# Autodesk Inventor assembly: Tolva
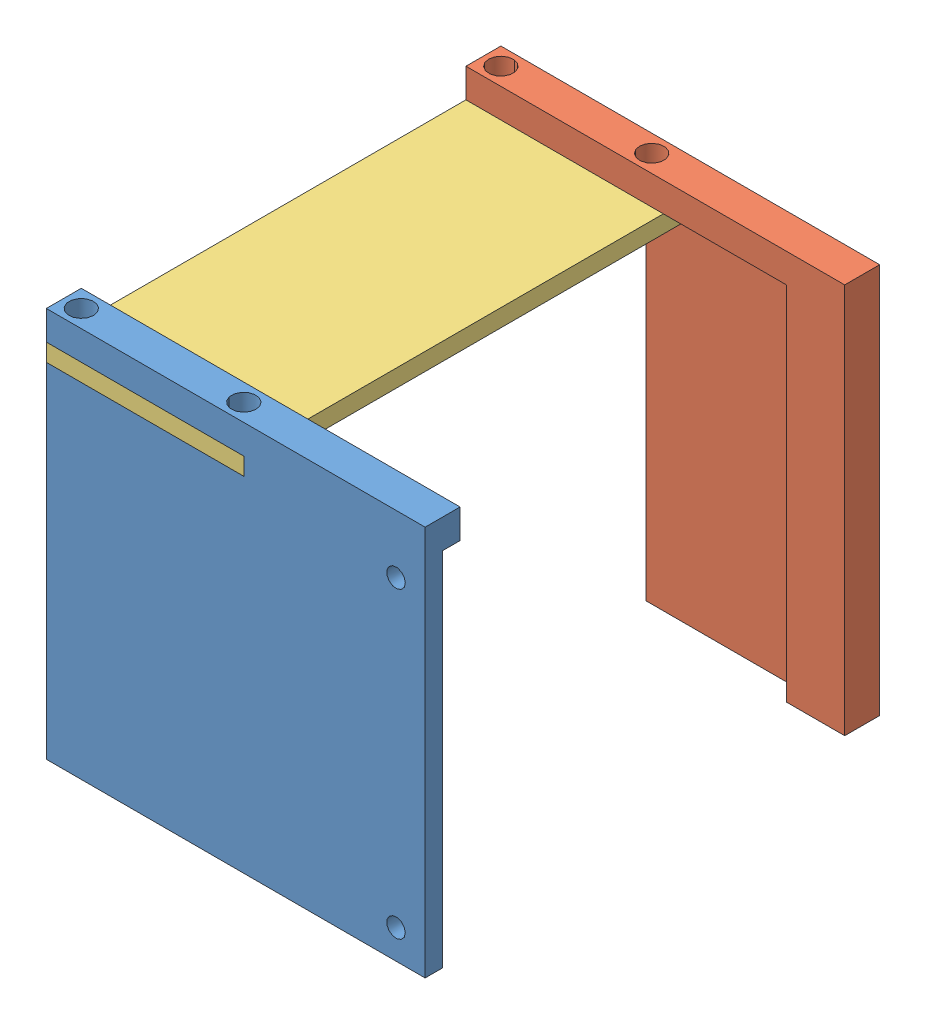
[picture p0: shaded view drawn from the part files that the assembly names]
Saved by Autodesk Inventor 2024 (Build 280153000, 153)
## iProperties
Created: 2025-03-02
Part Number: Tolva
Document SubType Name: Assembly
Designer: sergi
Author: sergi
## Documents named in this file (4)
- C:\Users\sergi\OneDrive\Escritorio\Projects\16. Protection catapult\Inventor\Tolva.iam
- C:\Users\sergi\OneDrive\Escritorio\Projects\16. Protection catapult\Inventor\Lateral izquierdo.ipt
- C:\Users\sergi\OneDrive\Escritorio\Projects\16. Protection catapult\Inventor\Lateral trasero.ipt
- C:\Users\sergi\OneDrive\Escritorio\Projects\16. Protection catapult\Inventor\Lateral derecho.ipt
## Components (3 placed, 3 different names)
1. Lateral izquierdo:1 — Coincidencia:1, Nivelación:1, Nivelación:2, Nivelación:3, Nivelación:4
2. Lateral derecho:1 — Nivelación:3, Nivelación:4, Nivelación:5
3. Lateral trasero:1 — Coincidencia:1, Nivelación:1, Nivelación:2, Nivelación:5
## Relationships (6: Flush 5, Mate 1)
- Coincidencia:1 [Mate]: Lateral izquierdo:1 ↔ Lateral trasero:1
- Nivelación:1 [Flush]: Lateral izquierdo:1 ↔ Lateral trasero:1
- Nivelación:2 [Flush]: Lateral izquierdo:1 ↔ Lateral trasero:1
- Nivelación:3 [Flush]: Lateral izquierdo:1 ↔ Lateral derecho:1
- Nivelación:4 [Flush]: Lateral izquierdo:1 ↔ Lateral derecho:1
- Nivelación:5 [Flush]: Lateral derecho:1 ↔ Lateral trasero:1
